# Autodesk Inventor assembly: Assembly_4DOF
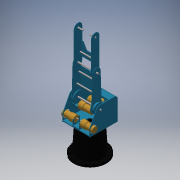
[picture p0: Inventor's stored thumbnail of the model, 180x180]
Saved by Autodesk Inventor 2016 (Build 200138000, 138)
## iProperties
Created: 2015-05-19
Part Number: Assembly_4DOF
Document SubType Name: Assembly
Designer: CHUNGBK
Author: CHUNGBK
## Documents named in this file (6)
- C:\Users\jonathan\Desktop\Five Axis Serial Robotic Arm\Inventor\Scorbot 3DOF.iam
- C:\Users\jonathan\Desktop\Five Axis Serial Robotic Arm\Inventor\Scorbot Platform.iam
- C:\Users\jonathan\Desktop\Five Axis Serial Robotic Arm\Inventor\Scorbot Shoulder.iam
- C:\Users\jonathan\Desktop\Five Axis Serial Robotic Arm\Inventor\Scorbot Elbow.iam
- C:\Users\jonathan\Desktop\Five Axis Serial Robotic Arm\Inventor\Motor Shaft.ipt
- C:\Users\jonathan\Desktop\Five Axis Serial Robotic Arm\Inventor\Base.ipt
## Components (9 placed, 5 different names)
1. Scorbot Platform:1 [sub-assembly] — Mate:1, Mate:2, Mate:4, Mate:5, Mate:6, Mate:7, Mate:8, Mate:9, Mate:10, Mate:11, Mate:12, Mate:13, Mate:27, Mate:28, Angle:1, Angle:2, Angle:4
2. Scorbot Shoulder:1 [sub-assembly] — Mate:1, Mate:2, Mate:3, Flush:5, Angle:4
3. Scorbot Elbow:1 [sub-assembly] — Mate:3, Flush:5, Angle:2
4. Motor Shaft:1 — Mate:4, Mate:5
5. Motor Shaft:2 — Mate:7, Mate:12
6. Motor Shaft:3 — Mate:8, Mate:13
7. Motor Shaft:4 — Mate:9, Mate:10
8. Motor Shaft:5 — Mate:6, Mate:11
9. Base:1 — Flush:6, Flush:7, Flush:8, Mate:27, Mate:28
## Relationships (22: Mate 15, Flush 4, Angle 3)
- Mate:1: Scorbot Platform:1 ↔ Scorbot Shoulder:1
- Mate:2 (23.3997 mm): Scorbot Platform:1 ↔ Scorbot Shoulder:1
- Mate:3: Scorbot Shoulder:1 ↔ Scorbot Elbow:1
- Flush:5 (8.7313 mm): Scorbot Shoulder:1 ↔ Scorbot Elbow:1
- Mate:4: Scorbot Platform:1 ↔ Motor Shaft:1
- Mate:5 (-19.05 mm): Scorbot Platform:1 ↔ Motor Shaft:1
- Mate:6: Scorbot Platform:1 ↔ Motor Shaft:5
- Mate:7: Scorbot Platform:1 ↔ Motor Shaft:2
- Mate:8: Scorbot Platform:1 ↔ Motor Shaft:3
- Mate:9: Scorbot Platform:1 ↔ Motor Shaft:4
- Mate:10 (-19.05 mm): Scorbot Platform:1 ↔ Motor Shaft:4
- Mate:11 (19.05 mm): Scorbot Platform:1 ↔ Motor Shaft:5
- Mate:12 (-19.05 mm): Scorbot Platform:1 ↔ Motor Shaft:2
- Mate:13 (-19.05 mm): Scorbot Platform:1 ↔ Motor Shaft:3
- Flush:6: Base:1
- Flush:7: Base:1
- Flush:8: Base:1
- Mate:27: Scorbot Platform:1 ↔ Base:1
- Mate:28 (23.8125 mm): Scorbot Platform:1 ↔ Base:1
- Angle:1 (0 deg): Scorbot Platform:1
- Angle:2 (0 deg): Scorbot Platform:1 ↔ Scorbot Elbow:1
- Angle:4 (0 deg): Scorbot Platform:1 ↔ Scorbot Shoulder:1
